# Autodesk Inventor assembly: ChessBoard
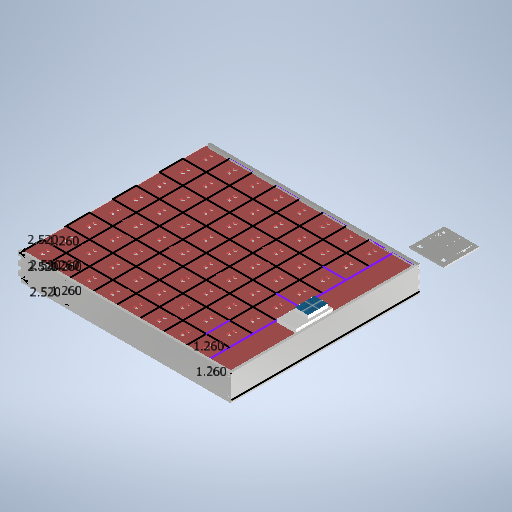
[picture p0: Inventor's stored thumbnail of the model, 512x512]
Saved by Autodesk Inventor 2025.2 (Build 292293000, 293)
## iProperties
Created: 2025-04-21
Part Number: ChessBoard
Document SubType Name: Assembly
Designer: powel
Author: powel
## Documents named in this file (8)
- C:\Users\powel\Desktop\School\24-25\Spring\Chess Set\ChessBoard.iam
- C:\Users\powel\Desktop\School\24-25\Spring\Chess Set\LED Holder.ipt
- C:\Users\powel\Desktop\School\24-25\Spring\Chess Set\Side Wall.ipt
- C:\Users\powel\Desktop\School\24-25\Spring\Chess Set\Floor.ipt
- C:\Users\powel\Desktop\School\24-25\Spring\Chess Set\Side Wall 3.ipt
- C:\Users\powel\Desktop\School\24-25\Spring\Chess Set\Wire Position.ipt
- C:\Users\powel\Desktop\School\24-25\Spring\Chess Set\LED Position.ipt
- C:\Users\powel\Desktop\School\24-25\Spring\Chess Set\Wall Test.ipt
## Components (9 placed, 7 different names)
1. LED Holder:1 — Rigid:3
2. Side Wall:1 — Rigid:1, Rigid:2, Rigid:3, Rigid:4
3. Floor:1 — Rigid:4
4. Floor:2 — Rigid:1
5. Side Wall 3:1 — Rigid:2, Rigid:5
6. Wire Position:1
7. LED Position:1
8. Wall Test:1
9. Side Wall:2 — Rigid:5
## Relationships (5: WeldJoint 5)
- Rigid:1 [WeldJoint]: Side Wall:1 ↔ Floor:2
- Rigid:2 [WeldJoint]: Side Wall:1 ↔ Side Wall 3:1
- Rigid:3 [WeldJoint]: LED Holder:1 ↔ Side Wall:1
- Rigid:4 [WeldJoint]: Side Wall:1 ↔ Floor:1
- Rigid:5 [WeldJoint]: Side Wall 3:1 ↔ Side Wall:2
## Named parameters: Finish11_Area = 1995.62, Finish1_Area = 3267.73, Finish2_Area = 5.06317, Finish3_Area = 20.1946, Finish4_Area = 1502.2, Finish5_Area = 232.393, Finish6_Area = 1509.57, Finish7_Area = 5.06317, Finish8_Area = 20.1946, Finish9_Area = 1502.2
note: some values were not read from the file. Shown as the stored number, unit unknown: "Finish11_Area", "Finish1_Area", "Finish2_Area", "Finish3_Area", "Finish4_Area", "Finish5_Area", "Finish6_Area", "Finish7_Area", "Finish8_Area", "Finish9_Area".
